# Autodesk Inventor assembly: DPLX_A002_Lab_Version
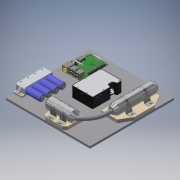
[picture p0: Inventor's stored thumbnail of the model, 180x180]
Saved by Autodesk Inventor 2018 (Build 220112000, 112)
## iProperties
Created: 2018-06-11
Part Number: DPLX_A002_Lab_Version
Document SubType Name: Assembly
Designer: DPLXuser
Author: DPLXuser
## Documents named in this file (8)
- C:\Users\DPLXuser\Documents\Michael Schwab\New folder\DPLX_A002_Lab_Version.iam
- C:\Users\DPLXuser\Documents\Michael Schwab\New folder\DPLX_P013_Lab_Baseplate.ipt
- C:\Users\DPLXuser\Documents\Michael Schwab\Aether PacknGo 6-4-18 8PM\SSL Spark Gap with Insulation.iam
- C:\Users\DPLXuser\Documents\Michael Schwab\Aether PacknGo 6-4-18 8PM\SSL VIPE Insulated Mount.iam
- C:\Users\DPLXuser\Documents\Michael Schwab\Aether PacknGo 6-4-18 8PM\Ocean Optics Flame.iam
- C:\Users\DPLXuser\Documents\Michael Schwab\Aether PacknGo 6-4-18 8PM\RPS 4 Battery mount.iam
- C:\Users\DPLXuser\Documents\Michael Schwab\Aether PacknGo 6-4-18 8PM\RPi3.iam
- C:\Users\DPLXuser\Documents\Michael Schwab\New folder\Wire3.ipt
## Components (7 placed, 7 different names)
1. DPLX_P013_Lab_Baseplate:1 — Mate:1, Mate:2, Mate:3, Mate:4, Mate:5, Mate:6, Mate:8, Mate:9, Mate:10, Flush:1, Flush:2
2. SSL Spark Gap with Insulation:1 [sub-assembly] — Mate:1, Mate:2, Mate:7, Mate:12, Flush:5
3. SSL VIPE Insulated Mount:1 [sub-assembly] — Mate:3, Mate:4, Mate:11, Flush:4
4. Ocean Optics Flame:1 [sub-assembly] — Mate:5, Mate:6, Mate:7
5. RPS 4 Battery mount:1 [sub-assembly] — Mate:8, Mate:9
6. RPi3:1 [sub-assembly] — Mate:10, Flush:1, Flush:2, Mate:13
7. Wire3:1 — Flush:3, Flush:4, Flush:5, Flush:6
## Relationships (19: Mate 13, Flush 6)
- Mate:1: DPLX_P013_Lab_Baseplate:1 ↔ SSL Spark Gap with Insulation:1
- Mate:2 (25.4 mm): DPLX_P013_Lab_Baseplate:1 ↔ SSL Spark Gap with Insulation:1
- Mate:3 (1.524 mm): DPLX_P013_Lab_Baseplate:1 ↔ SSL VIPE Insulated Mount:1
- Mate:4 (76.2 mm): DPLX_P013_Lab_Baseplate:1 ↔ SSL VIPE Insulated Mount:1
- Mate:5: DPLX_P013_Lab_Baseplate:1 ↔ Ocean Optics Flame:1
- Mate:6 (64.262 mm): DPLX_P013_Lab_Baseplate:1 ↔ Ocean Optics Flame:1
- Mate:7 (25.4 mm): SSL Spark Gap with Insulation:1 ↔ Ocean Optics Flame:1
- Mate:8: DPLX_P013_Lab_Baseplate:1 ↔ RPS 4 Battery mount:1
- Mate:9: DPLX_P013_Lab_Baseplate:1 ↔ RPS 4 Battery mount:1
- Mate:10: DPLX_P013_Lab_Baseplate:1 ↔ RPi3:1
- Flush:1 (12.7 mm): DPLX_P013_Lab_Baseplate:1 ↔ RPi3:1
- Flush:2 (12.7 mm): DPLX_P013_Lab_Baseplate:1 ↔ RPi3:1
- Mate:11: SSL VIPE Insulated Mount:1
- Mate:12: SSL Spark Gap with Insulation:1
- Mate:13: RPi3:1
- Flush:3: Wire3:1
- Flush:4: SSL VIPE Insulated Mount:1 ↔ Wire3:1
- Flush:5: SSL Spark Gap with Insulation:1 ↔ Wire3:1
- Flush:6: Wire3:1
